# Autodesk Inventor assembly: Anemometer Assy
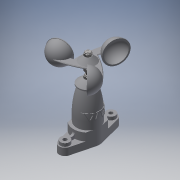
[picture p0: Inventor's stored thumbnail of the model, 180x180]
Saved by Autodesk Inventor 2019 (Build 230136000, 136)
## iProperties
Created: 2020-01-30
Part Number: Anemometer Assy
Document SubType Name: Assembly
Designer: alb16148
Author: alb16148
## Documents named in this file (11)
- N:\Sandpit\Callum Brooksby\anenometer\Anemometer Assy.iam
- N:\Sandpit\Callum Brooksby\anenometer\Base.ipt
- N:\Sandpit\Callum Brooksby\anenometer\Lid.ipt
- N:\Sandpit\Callum Brooksby\anenometer\Cap.ipt
- N:\Sandpit\Callum Brooksby\anenometer\Main Rod.ipt
- N:\Sandpit\Callum Brooksby\anenometer\Scoops.ipt
- N:\Sandpit\Callum Brooksby\anenometer\626-2rs\inafag_626-2rs.iam
- N:\Sandpit\Callum Brooksby\anenometer\M6 K-Nut Short.ipt
- N:\Sandpit\Callum Brooksby\anenometer\M6 Nut Plain.ipt
- N:\Sandpit\Callum Brooksby\anenometer\Bottom.ipt
- N:\Sandpit\Callum Brooksby\anenometer\Disk-3.ipt
## Components (16 placed, 10 different names)
1. Base:1 — Insert:1, Insert:5, Mate:2, Mate:3, Mate:4
2. Lid:1 — Insert:1, Insert:2, Insert:4
3. Cap:1 — Insert:2, Insert:12
4. Main Rod:1 — Insert:3
5. Scoops:1 — Insert:3, Insert:10, Insert:11
6. inafag_626-2rs:1 [sub-assembly] — Insert:4, Insert:6
7. inafag_626-2rs:2 [sub-assembly] — Insert:5, Insert:7, Insert:8
8. M6 K-Nut Short:1 — Insert:7
9. M6 K-Nut Short:2 — Insert:6
10. M6 K-Nut Short:3 — Insert:10
11. M6 K-Nut Short:4 — Insert:11
12. M6 Nut Plain:1 — Insert:8, Insert:13
13. M6 Nut Plain:2 — Insert:14
14. M6 K-Nut Short:5 — Insert:12
15. Bottom:1 — Mate:2, Mate:3, Mate:4
16. Disk-3:1 — Insert:13, Insert:14
## Relationships (16: Insert 13, Mate 3)
- Insert:1: Base:1 ↔ Lid:1
- Insert:2 (1 mm): Lid:1 ↔ Cap:1
- Insert:3 (6 mm): Main Rod:1 ↔ Scoops:1
- Insert:4: Lid:1 ↔ inafag_626-2rs:1
- Insert:5: Base:1 ↔ inafag_626-2rs:2
- Insert:6: inafag_626-2rs:1 ↔ M6 K-Nut Short:2
- Insert:7: inafag_626-2rs:2 ↔ M6 K-Nut Short:1
- Insert:8: inafag_626-2rs:2 ↔ M6 Nut Plain:1
- Insert:10: Scoops:1 ↔ M6 K-Nut Short:3
- Insert:11: Scoops:1 ↔ M6 K-Nut Short:4
- Insert:12: Cap:1 ↔ M6 K-Nut Short:5
- Mate:2: Base:1 ↔ Bottom:1
- Mate:3: Base:1 ↔ Bottom:1
- Mate:4: Base:1 ↔ Bottom:1
- Insert:13: M6 Nut Plain:1 ↔ Disk-3:1
- Insert:14: M6 Nut Plain:2 ↔ Disk-3:1
